# Autodesk Inventor assembly: Assy_fork_right_left
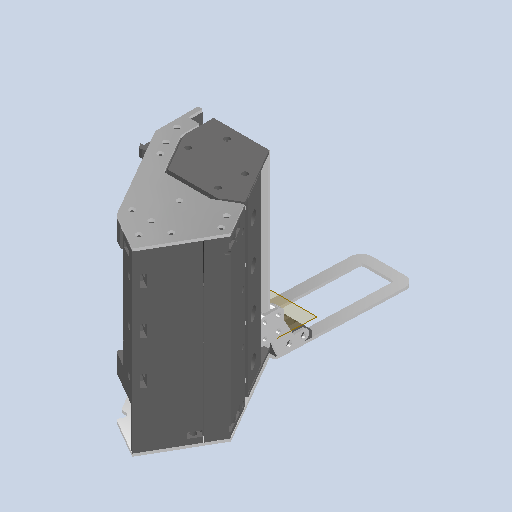
[picture p0: Inventor's stored thumbnail of the model, 512x512]
Saved by Autodesk Inventor 2024.1 (Build 281209000, 209)
## iProperties
Created: 2025-01-17
Part Number: Assy_fork_right_left
Document SubType Name: Assembly
Designer: hibik
Author: hibik
## Documents named in this file (4)
- C:\Users\hibik\Documents\Robomech\RESCUE\ORCA\hard\fork\left\Assy_fork_right_left.iam
- C:\Users\hibik\Documents\Robomech\RESCUE\ORCA\hard\fork\left\base_wall_added_left.iam
- C:\Users\hibik\Documents\Robomech\RESCUE\ORCA\hard\fork\left\screw_left.iam
- C:\Users\hibik\Documents\Robomech\RESCUE\ORCA\hard\fork\left\rail_left.iam
## Components (3 placed, 3 different names)
1. base_wall_added_left:1 [sub-assembly] — 挿入:3, 正接:3, 正接:2, 正接:1, 正接:4, 正接:5
2. screw_left:1 [sub-assembly] — 挿入:3
3. rail_left:1 [sub-assembly] — 正接:3, 正接:2, 正接:1, 正接:4, 正接:5
## Relationships (6: Tangent 5, Insert 1)
- 挿入:3 [Insert]: base_wall_added_left:1 ↔ screw_left:1
- 正接:3 [Tangent]: base_wall_added_left:1 ↔ rail_left:1
- 正接:2 [Tangent]: base_wall_added_left:1 ↔ rail_left:1
- 正接:1 [Tangent]: base_wall_added_left:1 ↔ rail_left:1
- 正接:4 [Tangent]: base_wall_added_left:1 ↔ rail_left:1
- 正接:5 [Tangent]: base_wall_added_left:1 ↔ rail_left:1
